# Autodesk Inventor assembly: MG-Straight Kicker
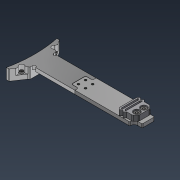
[picture p0: Inventor's stored thumbnail of the model, 180x180]
Saved by Autodesk Inventor 2022.1 (Build 261234020, 234B)
## iProperties
Part Number: MG-Straight Kicker
Material: Generisch
Document SubType Name: Assembly
Designer: rYan
Mass: 83.0853 g
Surface Area: 121.113 cm^2
Volume: 18.2277 cm^3
Density: 4.5582 g/cm^3
Author: rYan
## Documents named in this file (7)
- D:\TIGERsGIT\Hardware\mechanik\2020\Inventor\Robot\Kicker\MG-Straight Kicker.iam
- D:\TIGERsGIT\Hardware\mechanik\2020\Inventor\Robot\Kicker\Kicker Eisen.ipt
- D:\TIGERsGIT\Hardware\mechanik\2020\Inventor\Robot\Kicker\Kicker Sichel.ipt
- D:\TIGERsGIT\Hardware\mechanik\2020\Inventor\Inhaltscenter\de-DE\ISO 4762(2)\ISO 4762 - M2 x 6ISO.ipt
- D:\TIGERsGIT\Hardware\mechanik\2020\Inventor\Robot\Kicker\Kickerdaempfer.ipt
- D:\TIGERsGIT\Hardware\mechanik\2020\Inventor\Inhaltscenter\de-DE\DIN 7984\DIN 7984 - M4 x 6.ipt
- D:\TIGERsGIT\Hardware\mechanik\2020\Inventor\Purchased Parts\ISO 10642 - M3 x 4.ipt
## Components (11 placed, 6 different names)
1. Kicker Sichel:1 — Fluchtend:1, Fluchtend:2, Fluchtend:3, Einfügen:9, Einfügen:10, Einfügen:15, Passend:3, Einfügen:16, Einfügen:17, Einfügen:18, Einfügen:19
2. Kicker Eisen:1 — Einfügen:12, Passend:2, Einfügen:15, Passend:3
3. ISO 4762 M2 x 6:1 — Einfügen:9
4. ISO 4762 M2 x 6:2 — Einfügen:10
5. Kickerdaempfer:1 — Einfügen:12, Passend:2, Einfügen:13, Einfügen:14
6. DIN 7984 M4 x 6:1 — Einfügen:14
7. DIN 7984 M4 x 6:2 — Einfügen:13
8. ISO 10642 M3 x  6:2 — Einfügen:16
9. ISO 10642 M3 x  6:3 — Einfügen:19
10. ISO 10642 M3 x  6:4 — Einfügen:17
11. ISO 10642 M3 x  6:5 — Einfügen:18
## Relationships (15: Insert 10, Flush 3, Mate 2)
- Fluchtend:1 [Flush]: Kicker Sichel:1
- Fluchtend:2 [Flush]: Kicker Sichel:1
- Fluchtend:3 [Flush]: Kicker Sichel:1
- Einfügen:9 [Insert] (0.5 mm): Kicker Sichel:1 ↔ ISO 4762 M2 x 6:1
- Einfügen:10 [Insert] (0.5 mm): Kicker Sichel:1 ↔ ISO 4762 M2 x 6:2
- Einfügen:12 [Insert]: Kicker Eisen:1 ↔ Kickerdaempfer:1
- Passend:2 [Mate]: Kicker Eisen:1 ↔ Kickerdaempfer:1
- Einfügen:13 [Insert]: Kickerdaempfer:1 ↔ DIN 7984 M4 x 6:2
- Einfügen:14 [Insert]: Kickerdaempfer:1 ↔ DIN 7984 M4 x 6:1
- Einfügen:15 [Insert]: Kicker Sichel:1 ↔ Kicker Eisen:1
- Passend:3 [Mate]: Kicker Sichel:1 ↔ Kicker Eisen:1
- Einfügen:16 [Insert]: Kicker Sichel:1 ↔ ISO 10642 M3 x  6:2
- Einfügen:17 [Insert]: Kicker Sichel:1 ↔ ISO 10642 M3 x  6:4
- Einfügen:18 [Insert]: Kicker Sichel:1 ↔ ISO 10642 M3 x  6:5
- Einfügen:19 [Insert]: Kicker Sichel:1 ↔ ISO 10642 M3 x  6:3
